# Autodesk Inventor assembly: Tornillo Soinfin_v001
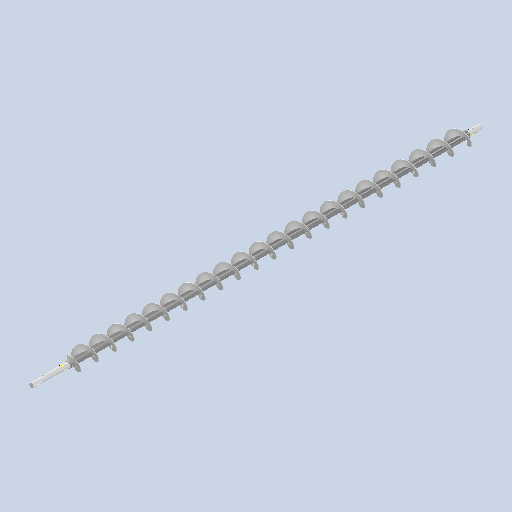
[picture p0: Inventor's stored thumbnail of the model, 512x512]
Saved by Autodesk Inventor 2024 (Build 280153000, 153)
## iProperties
RuleStatus: InUse
Created: 2026-01-08
Part Number: Tornillo Soinfin_v001
Document SubType Name: Assembly
Designer: eduso
Author: eduso
## Documents named in this file (6)
- C:\edusonros_projects\SINFINES_CONRAD\iLogic\Tornillo Soinfin_v001.iam
- C:\edusonros_projects\SINFINES_CONRAD\iLogic\Tubo_Perforado_Base.ipt
- C:\edusonros_projects\SINFINES_CONRAD\iLogic\Mangon_Conducido.ipt
- C:\edusonros_projects\SINFINES_CONRAD\iLogic\Mangon_Conduccion.ipt
- C:\edusonros_projects\SINFINES_CONRAD\iLogic\Espira_01.ipt
- C:\edusonros_projects\SINFINES_CONRAD\iLogic\Espira_01_Parcial.ipt
## Components (26 placed, 5 different names)
1. Tubo_Perforado_Base:1 — Mate:1, Mate:2, Mate:3, Mate:4, Mate:5, Mate:6
2. Mangon_Conducido:1 — Mate:1, Mate:2
3. Mangon_Conduccion:1 — Mate:3, Mate:4
4. Espira_01_Parcial:1 — Mate:7, Mate:8
5. Espira_01:1 — Mate:5, Mate:6
6. Espira_01:3
7. Espira_01:4
8. Espira_01:5
9. Espira_01:6
10. Espira_01:7
11. Espira_01:8
12. Espira_01:9
13. Espira_01:10
14. Espira_01:11
15. Espira_01:12
16. Espira_01:13
17. Espira_01:14
18. Espira_01:15
19. Espira_01:16
20. Espira_01:17
21. Espira_01:18
22. Espira_01:19
23. Espira_01:20
24. Espira_01:21
25. Espira_01:22
26. Espira_01:23 — Mate:7, Mate:8
## Component patterns: (22 elements, first: Espira_01:1)
## Relationships (8: Mate 8)
- Mate:1: Tubo_Perforado_Base:1 ↔ Mangon_Conducido:1
- Mate:2: Tubo_Perforado_Base:1 ↔ Mangon_Conducido:1
- Mate:3: Tubo_Perforado_Base:1 ↔ Mangon_Conduccion:1
- Mate:4: Tubo_Perforado_Base:1 ↔ Mangon_Conduccion:1
- Mate:5: Tubo_Perforado_Base:1 ↔ Espira_01:1
- Mate:6: Tubo_Perforado_Base:1 ↔ Espira_01:1
- Mate:7: Espira_01_Parcial:1 ↔ Espira_01:23
- Mate:8: Espira_01_Parcial:1 ↔ Espira_01:23
## Named parameters: Paso_Espira_01 = 200 mm, ø_Ext_Espira_01 = 200 mm, ø_Int_Espira_01 = 60.3 mm, Espesor_Espira_01 = 6 mm, Testero_007 = 4 mm, Espacio_008 = 50 mm, Inteerior_Tubo_009 = 80 mm, Cido_Testero_007 = 4 mm, Cido_Espacio_008 = 50 mm, Cido_Inteerior_Tubo_009 = 80 mm, Largo = 4500 mm, DiametroExterior = 70 mm, Espesor = 6 mm, DiametroInterior = 58 mm, Num_Espiras = 22, Resto = 100 mm
